# Autodesk Inventor assembly: hot box
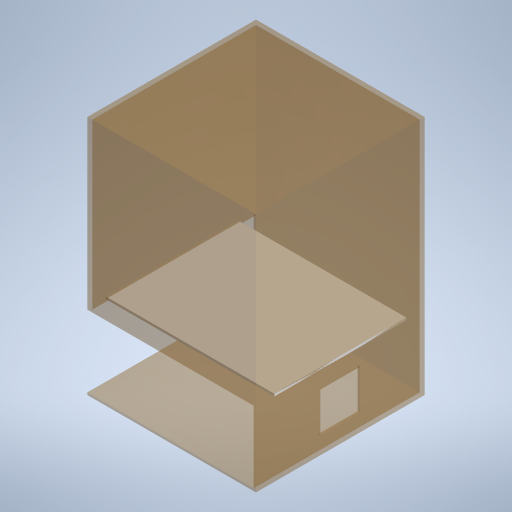
[picture p0: Inventor's stored thumbnail of the model, 512x512]
Saved by Autodesk Inventor 2023 (Build 270158000, 158)
## iProperties
Created: 2022-08-07
Part Number: hot box
Document SubType Name: Assembly
Designer: techv
Author: techv
## Documents named in this file (3)
- D:\Projects\P_Baker Bot\Design\STL\hot box.iam
- D:\Projects\P_Baker Bot\Design\STL\Hot Box Case.ipt
- D:\Projects\P_Baker Bot\Design\STL\Baffle.ipt
## Components (2 placed, 2 different names)
1. Hot Box Case:1 — Flush:1, Flush:2
2. Baffle:1 — Flush:1, Flush:2
## Relationships (2: Flush 2)
- Flush:1: Hot Box Case:1 ↔ Baffle:1
- Flush:2: Hot Box Case:1 ↔ Baffle:1
